# Autodesk Inventor assembly: 110033226_iam_12_船屋
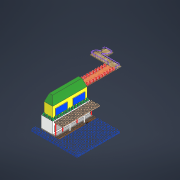
[picture p0: Inventor's stored thumbnail of the model, 180x180]
Saved by Autodesk Inventor 2022 (Build 260153000, 153)
## iProperties
Created: 2022-06-28
Part Number: 110033226_iam_12_船屋
Document SubType Name: Assembly
Designer: User
Author: User
## Documents named in this file (7)
- D:\D-disk\pomelo\大一\下學期\機械設計製圖\1100332260_LEGOproj_沒有公主城堡\110033226_iam_12_船屋.iam
- D:\D-disk\pomelo\大一\下學期\機械設計製圖\1100332260_LEGOproj_沒有公主城堡\110033226_ipt_47_船屋基地.ipt
- D:\D-disk\pomelo\大一\下學期\機械設計製圖\1100332260_LEGOproj_沒有公主城堡\110033226_ipt_48_船屋梁架.ipt
- D:\D-disk\pomelo\大一\下學期\機械設計製圖\1100332260_LEGOproj_沒有公主城堡\110033226_ipt_49_船屋主體.ipt
- D:\D-disk\pomelo\大一\下學期\機械設計製圖\1100332260_LEGOproj_沒有公主城堡\110033226_ipt_50_船屋圓柱.ipt
- D:\D-disk\pomelo\大一\下學期\機械設計製圖\1100332260_LEGOproj_沒有公主城堡\110033226_ipt_21_柵欄.ipt
- D:\D-disk\pomelo\大一\下學期\機械設計製圖\1100332260_LEGOproj_沒有公主城堡\110033226_ipt_04_小河.ipt
## Components (353 placed, 6 different names)
1. 110033226_ipt_48_船屋梁架:1 — 貼合:4, 貼合:5, 貼合:7
2. 110033226_ipt_49_船屋主體:1 — 貼合:6, 貼合:7, 貼合:11, 貼合:12, 貼合:13, 貼合:14, 貼合:15, 貼合:16, 貼合:17, 貼合:18, 貼合:19, 貼合:20, 貼合:21, 貼合:22, 貼合:23, 貼合:24, 貼合:25, 貼合:26, 貼合:27, 貼合:28, 貼合:29, 貼合:30, 貼合:31, 貼合:32, 貼合:33, 貼合:34
3. 110033226_ipt_21_柵欄:32 — 貼合:27, 貼合:28, 貼合:29, 角度:1
4. 110033226_ipt_47_船屋基地:1 — 貼合:1, 貼合:2, 貼合:3, 貼合:35, 貼合:36, 貼合:37, 貼合:38, 貼合:39, 貼合:40
5. 110033226_ipt_47_船屋基地:2 — 貼合:4, 貼合:5, 貼合:6, 貼合:8, 貼合:9, 貼合:10, 貼合:13, 貼合:14
6. 110033226_ipt_50_船屋圓柱:1 — 貼合:8, 貼合:9, 貼合:10
7. 110033226_ipt_50_船屋圓柱:2
8. 110033226_ipt_21_柵欄:1 — 貼合:11, 貼合:12
9. 110033226_ipt_21_柵欄:2
10. 110033226_ipt_21_柵欄:3
11. 110033226_ipt_21_柵欄:4
12. 110033226_ipt_21_柵欄:5
13. 110033226_ipt_21_柵欄:6
14. 110033226_ipt_21_柵欄:7
15. 110033226_ipt_21_柵欄:8
16. 110033226_ipt_21_柵欄:9
17. 110033226_ipt_21_柵欄:10
18. 110033226_ipt_21_柵欄:11
19. 110033226_ipt_21_柵欄:12
20. 110033226_ipt_21_柵欄:13
21. 110033226_ipt_21_柵欄:14 — 貼合:15, 貼合:16, 貼合:17
22. 110033226_ipt_21_柵欄:15
23. 110033226_ipt_21_柵欄:16
24. 110033226_ipt_21_柵欄:17
25. 110033226_ipt_21_柵欄:18
26. 110033226_ipt_21_柵欄:19
27. 110033226_ipt_21_柵欄:21 — 貼合:18, 貼合:19, 貼合:20
28. 110033226_ipt_21_柵欄:23
29. 110033226_ipt_21_柵欄:22 — 貼合:21, 貼合:22, 貼合:23
30. 110033226_ipt_21_柵欄:24
31. 110033226_ipt_21_柵欄:25
32. 110033226_ipt_21_柵欄:26
33. 110033226_ipt_21_柵欄:27
34. 110033226_ipt_21_柵欄:20 — 貼合:24, 貼合:25, 貼合:26
35. 110033226_ipt_21_柵欄:28
36. 110033226_ipt_21_柵欄:29
37. 110033226_ipt_21_柵欄:30
38. 110033226_ipt_21_柵欄:31 — 貼合:30, 貼合:31, 角度:1
39. 110033226_ipt_21_柵欄:33
40. 110033226_ipt_21_柵欄:34
41. 110033226_ipt_21_柵欄:35
42. 110033226_ipt_21_柵欄:36
43. 110033226_ipt_21_柵欄:37
44. 110033226_ipt_21_柵欄:38
45. 110033226_ipt_21_柵欄:39
46. 110033226_ipt_21_柵欄:40
47. 110033226_ipt_21_柵欄:41
48. 110033226_ipt_21_柵欄:42
49. 110033226_ipt_21_柵欄:43
50. 110033226_ipt_21_柵欄:44
51. 110033226_ipt_21_柵欄:45
52. 110033226_ipt_21_柵欄:46
53. 110033226_ipt_21_柵欄:47
54. 110033226_ipt_21_柵欄:48
55. 110033226_ipt_21_柵欄:49 — 貼合:32, 貼合:33, 貼合:34
56. 110033226_ipt_21_柵欄:50
57. 110033226_ipt_21_柵欄:51
58. 110033226_ipt_21_柵欄:52
59. 110033226_ipt_21_柵欄:53
60. 110033226_ipt_21_柵欄:54
61. 110033226_ipt_21_柵欄:55
62. 110033226_ipt_21_柵欄:56
63. 110033226_ipt_21_柵欄:57
64. 110033226_ipt_21_柵欄:58
65. 110033226_ipt_21_柵欄:59
66. 110033226_ipt_21_柵欄:60
67. 110033226_ipt_21_柵欄:61
68. 110033226_ipt_21_柵欄:62
69. 110033226_ipt_21_柵欄:63
70. 110033226_ipt_21_柵欄:64
71. 110033226_ipt_21_柵欄:65
72. 110033226_ipt_21_柵欄:66
73. 110033226_ipt_21_柵欄:67
74. 110033226_ipt_04_小河:2 — 貼合:36, 貼合:39, 貼合:40
75. 110033226_ipt_04_小河:29
76. 110033226_ipt_04_小河:30
77. 110033226_ipt_04_小河:31
78. 110033226_ipt_04_小河:32
79. 110033226_ipt_04_小河:33
80. 110033226_ipt_04_小河:34
81. 110033226_ipt_04_小河:35
82. 110033226_ipt_04_小河:36
83. 110033226_ipt_04_小河:37
84. 110033226_ipt_04_小河:38
85. 110033226_ipt_04_小河:39
86. 110033226_ipt_04_小河:40
87. 110033226_ipt_04_小河:41
88. 110033226_ipt_04_小河:42
89. 110033226_ipt_04_小河:43
90. 110033226_ipt_04_小河:44
91. 110033226_ipt_04_小河:45
92. 110033226_ipt_04_小河:46
93. 110033226_ipt_04_小河:47
94. 110033226_ipt_04_小河:48
95. 110033226_ipt_04_小河:49
96. 110033226_ipt_04_小河:50
97. 110033226_ipt_04_小河:51
98. 110033226_ipt_04_小河:52
99. 110033226_ipt_04_小河:53
100. 110033226_ipt_04_小河:54
101. 110033226_ipt_04_小河:55
102. 110033226_ipt_04_小河:56
103. 110033226_ipt_04_小河:57
104. 110033226_ipt_04_小河:58
105. 110033226_ipt_04_小河:59
106. 110033226_ipt_04_小河:60
107. 110033226_ipt_04_小河:61
108. 110033226_ipt_04_小河:62
109. 110033226_ipt_04_小河:63
110. 110033226_ipt_04_小河:64
111. 110033226_ipt_04_小河:65
112. 110033226_ipt_04_小河:66
113. 110033226_ipt_04_小河:67
114. 110033226_ipt_04_小河:68
115. 110033226_ipt_04_小河:69
116. 110033226_ipt_04_小河:70
117. 110033226_ipt_04_小河:71
118. 110033226_ipt_04_小河:72
119. 110033226_ipt_04_小河:73
120. 110033226_ipt_04_小河:74
121. 110033226_ipt_04_小河:75
122. 110033226_ipt_04_小河:76
123. 110033226_ipt_04_小河:77
124. 110033226_ipt_04_小河:78
125. 110033226_ipt_04_小河:79
126. 110033226_ipt_04_小河:80
127. 110033226_ipt_04_小河:81
128. 110033226_ipt_04_小河:82
129. 110033226_ipt_04_小河:83
130. 110033226_ipt_04_小河:84
131. 110033226_ipt_04_小河:85
132. 110033226_ipt_04_小河:86
133. 110033226_ipt_04_小河:87
134. 110033226_ipt_04_小河:88
135. 110033226_ipt_04_小河:89
136. 110033226_ipt_04_小河:90
137. 110033226_ipt_04_小河:91
138. 110033226_ipt_04_小河:1 — 貼合:35, 貼合:37, 貼合:38
139. 110033226_ipt_04_小河:3
140. 110033226_ipt_04_小河:4
141. 110033226_ipt_04_小河:5
142. 110033226_ipt_04_小河:6
143. 110033226_ipt_04_小河:7
144. 110033226_ipt_04_小河:8
145. 110033226_ipt_04_小河:9
146. 110033226_ipt_04_小河:10
147. 110033226_ipt_04_小河:11
148. 110033226_ipt_04_小河:12
149. 110033226_ipt_04_小河:13
150. 110033226_ipt_04_小河:14
151. 110033226_ipt_04_小河:15
152. 110033226_ipt_04_小河:16
153. 110033226_ipt_04_小河:17
154. 110033226_ipt_04_小河:18
155. 110033226_ipt_04_小河:19
156. 110033226_ipt_04_小河:20
157. 110033226_ipt_04_小河:21
158. 110033226_ipt_04_小河:22
159. 110033226_ipt_04_小河:23
160. 110033226_ipt_04_小河:24
161. 110033226_ipt_04_小河:25
162. 110033226_ipt_04_小河:26
163. 110033226_ipt_04_小河:27
164. 110033226_ipt_04_小河:28
165. 110033226_ipt_04_小河:92
166. 110033226_ipt_04_小河:93
167. 110033226_ipt_04_小河:94
168. 110033226_ipt_04_小河:95
169. 110033226_ipt_04_小河:96
170. 110033226_ipt_04_小河:97
171. 110033226_ipt_04_小河:98
172. 110033226_ipt_04_小河:99
173. 110033226_ipt_04_小河:100
174. 110033226_ipt_04_小河:101
175. 110033226_ipt_04_小河:102
176. 110033226_ipt_04_小河:103
177. 110033226_ipt_04_小河:104
178. 110033226_ipt_04_小河:105
179. 110033226_ipt_04_小河:106
180. 110033226_ipt_04_小河:107
181. 110033226_ipt_04_小河:108
182. 110033226_ipt_04_小河:109
183. 110033226_ipt_04_小河:110
184. 110033226_ipt_04_小河:111
185. 110033226_ipt_04_小河:112
186. 110033226_ipt_04_小河:113
187. 110033226_ipt_04_小河:114
188. 110033226_ipt_04_小河:115
189. 110033226_ipt_04_小河:116
190. 110033226_ipt_04_小河:117
191. 110033226_ipt_04_小河:118
192. 110033226_ipt_04_小河:119
193. 110033226_ipt_04_小河:120
194. 110033226_ipt_04_小河:121
195. 110033226_ipt_04_小河:122
196. 110033226_ipt_04_小河:123
197. 110033226_ipt_04_小河:124
198. 110033226_ipt_04_小河:125
199. 110033226_ipt_04_小河:126
200. 110033226_ipt_04_小河:127
201. 110033226_ipt_04_小河:128
202. 110033226_ipt_04_小河:129
203. 110033226_ipt_04_小河:130
204. 110033226_ipt_04_小河:131
205. 110033226_ipt_04_小河:132
206. 110033226_ipt_04_小河:133
207. 110033226_ipt_04_小河:134
208. 110033226_ipt_04_小河:135
209. 110033226_ipt_04_小河:136
210. 110033226_ipt_04_小河:137
211. 110033226_ipt_04_小河:138
212. 110033226_ipt_04_小河:139
213. 110033226_ipt_04_小河:140
214. 110033226_ipt_04_小河:141
215. 110033226_ipt_04_小河:142
216. 110033226_ipt_04_小河:143
217. 110033226_ipt_04_小河:144
218. 110033226_ipt_04_小河:145
219. 110033226_ipt_04_小河:146
220. 110033226_ipt_04_小河:147
221. 110033226_ipt_04_小河:148
222. 110033226_ipt_04_小河:149
223. 110033226_ipt_04_小河:150
224. 110033226_ipt_04_小河:151
225. 110033226_ipt_04_小河:152
226. 110033226_ipt_04_小河:153
227. 110033226_ipt_04_小河:154
228. 110033226_ipt_04_小河:155
229. 110033226_ipt_04_小河:156
230. 110033226_ipt_04_小河:157
231. 110033226_ipt_04_小河:158
232. 110033226_ipt_04_小河:159
233. 110033226_ipt_04_小河:160
234. 110033226_ipt_04_小河:161
235. 110033226_ipt_04_小河:162
236. 110033226_ipt_04_小河:163
237. 110033226_ipt_04_小河:164
238. 110033226_ipt_04_小河:165
239. 110033226_ipt_04_小河:166
240. 110033226_ipt_04_小河:167
241. 110033226_ipt_04_小河:168
242. 110033226_ipt_04_小河:169
243. 110033226_ipt_04_小河:170
244. 110033226_ipt_04_小河:171
245. 110033226_ipt_04_小河:172
246. 110033226_ipt_04_小河:173
247. 110033226_ipt_04_小河:174
248. 110033226_ipt_04_小河:175
249. 110033226_ipt_04_小河:176
250. 110033226_ipt_04_小河:177
251. 110033226_ipt_04_小河:178
252. 110033226_ipt_04_小河:179
253. 110033226_ipt_04_小河:180
254. 110033226_ipt_04_小河:181
255. 110033226_ipt_04_小河:182
256. 110033226_ipt_04_小河:183
257. 110033226_ipt_04_小河:184
258. 110033226_ipt_04_小河:185
259. 110033226_ipt_04_小河:186
260. 110033226_ipt_04_小河:187
261. 110033226_ipt_04_小河:188
262. 110033226_ipt_04_小河:189
263. 110033226_ipt_04_小河:190
264. 110033226_ipt_04_小河:191
265. 110033226_ipt_04_小河:192
266. 110033226_ipt_04_小河:193
267. 110033226_ipt_04_小河:194
268. 110033226_ipt_04_小河:195
269. 110033226_ipt_04_小河:196
270. 110033226_ipt_04_小河:197
271. 110033226_ipt_04_小河:198
272. 110033226_ipt_04_小河:199
273. 110033226_ipt_04_小河:200
274. 110033226_ipt_04_小河:201
275. 110033226_ipt_04_小河:202
276. 110033226_ipt_04_小河:203
277. 110033226_ipt_04_小河:204
278. 110033226_ipt_04_小河:205
279. 110033226_ipt_04_小河:206
280. 110033226_ipt_04_小河:207
281. 110033226_ipt_04_小河:208
282. 110033226_ipt_04_小河:209
283. 110033226_ipt_04_小河:210
284. 110033226_ipt_04_小河:211
285. 110033226_ipt_04_小河:212
286. 110033226_ipt_04_小河:213
287. 110033226_ipt_04_小河:214
288. 110033226_ipt_04_小河:215
289. 110033226_ipt_04_小河:216
290. 110033226_ipt_04_小河:217
291. 110033226_ipt_04_小河:218
292. 110033226_ipt_04_小河:219
293. 110033226_ipt_04_小河:220
294. 110033226_ipt_04_小河:221
295. 110033226_ipt_04_小河:222
296. 110033226_ipt_04_小河:223
297. 110033226_ipt_04_小河:224
298. 110033226_ipt_04_小河:225
299. 110033226_ipt_04_小河:226
300. 110033226_ipt_04_小河:227
301. 110033226_ipt_04_小河:228
302. 110033226_ipt_04_小河:229
303. 110033226_ipt_04_小河:230
304. 110033226_ipt_04_小河:231
305. 110033226_ipt_04_小河:232
306. 110033226_ipt_04_小河:233
307. 110033226_ipt_04_小河:234
308. 110033226_ipt_04_小河:235
309. 110033226_ipt_04_小河:236
310. 110033226_ipt_04_小河:237
311. 110033226_ipt_04_小河:238
312. 110033226_ipt_04_小河:239
313. 110033226_ipt_04_小河:240
314. 110033226_ipt_04_小河:241
315. 110033226_ipt_04_小河:242
316. 110033226_ipt_04_小河:243
317. 110033226_ipt_04_小河:244
318. 110033226_ipt_04_小河:245
319. 110033226_ipt_04_小河:246
320. 110033226_ipt_04_小河:247
321. 110033226_ipt_04_小河:248
322. 110033226_ipt_04_小河:249
323. 110033226_ipt_04_小河:250
324. 110033226_ipt_04_小河:251
325. 110033226_ipt_04_小河:252
326. 110033226_ipt_04_小河:253
327. 110033226_ipt_04_小河:254
328. 110033226_ipt_04_小河:255
329. 110033226_ipt_04_小河:256
330. 110033226_ipt_04_小河:257
331. 110033226_ipt_04_小河:258
332. 110033226_ipt_04_小河:259
333. 110033226_ipt_04_小河:260
334. 110033226_ipt_04_小河:261
335. 110033226_ipt_04_小河:262
336. 110033226_ipt_04_小河:263
337. 110033226_ipt_04_小河:264
338. 110033226_ipt_04_小河:265
339. 110033226_ipt_04_小河:266
340. 110033226_ipt_04_小河:267
341. 110033226_ipt_04_小河:268
342. 110033226_ipt_04_小河:269
343. 110033226_ipt_04_小河:270
344. 110033226_ipt_04_小河:271
345. 110033226_ipt_04_小河:272
346. 110033226_ipt_04_小河:273
347. 110033226_ipt_04_小河:274
348. 110033226_ipt_04_小河:275
349. 110033226_ipt_04_小河:276
350. 110033226_ipt_04_小河:277
351. 110033226_ipt_04_小河:278
352. 110033226_ipt_04_小河:279
353. 110033226_ipt_04_小河:280
## Component patterns: (2 elements, first: 110033226_ipt_47_船屋基地:1), (2 elements, first: 110033226_ipt_50_船屋圓柱:1), (13 elements, first: 110033226_ipt_21_柵欄:1), (6 elements, first: 110033226_ipt_21_柵欄:14), (2 elements, first: 110033226_ipt_21_柵欄:21), (5 elements, first: 110033226_ipt_21_柵欄:22), (4 elements, first: 110033226_ipt_21_柵欄:20), (17 elements, first: 110033226_ipt_21_柵欄:31), (19 elements, first: 110033226_ipt_21_柵欄:49), (2 elements), (8 elements), (32 elements, first: 110033226_ipt_04_小河:2), 元件陣列 11:2 (32 elements), (27 elements, first: 110033226_ipt_04_小河:1), 元件陣列 10:2 (27 elements), 元件陣列 10:3 (27 elements), 元件陣列 10:4 (27 elements), 元件陣列 10:5 (27 elements), 元件陣列 10:6 (27 elements), 元件陣列 10:7 (27 elements), 元件陣列 10:8 (27 elements)
## Relationships (41: Mate 40, Angle 1)
- 貼合:1 [Mate]: 110033226_ipt_47_船屋基地:1
- 貼合:2 [Mate]: 110033226_ipt_47_船屋基地:1
- 貼合:3 [Mate]: 110033226_ipt_47_船屋基地:1
- 貼合:4 [Mate]: 110033226_ipt_48_船屋梁架:1 ↔ 110033226_ipt_47_船屋基地:2
- 貼合:5 [Mate]: 110033226_ipt_48_船屋梁架:1 ↔ 110033226_ipt_47_船屋基地:2
- 貼合:6 [Mate]: 110033226_ipt_49_船屋主體:1 ↔ 110033226_ipt_47_船屋基地:2
- 貼合:7 [Mate]: 110033226_ipt_48_船屋梁架:1 ↔ 110033226_ipt_49_船屋主體:1
- 貼合:8 [Mate]: 110033226_ipt_47_船屋基地:2 ↔ 110033226_ipt_50_船屋圓柱:1
- 貼合:9 [Mate]: 110033226_ipt_47_船屋基地:2 ↔ 110033226_ipt_50_船屋圓柱:1
- 貼合:10 [Mate]: 110033226_ipt_47_船屋基地:2 ↔ 110033226_ipt_50_船屋圓柱:1
- 貼合:11 [Mate]: 110033226_ipt_49_船屋主體:1 ↔ 110033226_ipt_21_柵欄:1
- 貼合:12 [Mate]: 110033226_ipt_49_船屋主體:1 ↔ 110033226_ipt_21_柵欄:1
- 貼合:13 [Mate]: 110033226_ipt_49_船屋主體:1 ↔ 110033226_ipt_47_船屋基地:2
- 貼合:14 [Mate]: 110033226_ipt_49_船屋主體:1 ↔ 110033226_ipt_47_船屋基地:2
- 貼合:15 [Mate]: 110033226_ipt_49_船屋主體:1 ↔ 110033226_ipt_21_柵欄:14
- 貼合:16 [Mate]: 110033226_ipt_49_船屋主體:1 ↔ 110033226_ipt_21_柵欄:14
- 貼合:17 [Mate]: 110033226_ipt_49_船屋主體:1 ↔ 110033226_ipt_21_柵欄:14
- 貼合:18 [Mate]: 110033226_ipt_49_船屋主體:1 ↔ 110033226_ipt_21_柵欄:21
- 貼合:19 [Mate]: 110033226_ipt_49_船屋主體:1 ↔ 110033226_ipt_21_柵欄:21
- 貼合:20 [Mate]: 110033226_ipt_49_船屋主體:1 ↔ 110033226_ipt_21_柵欄:21
- 貼合:21 [Mate]: 110033226_ipt_49_船屋主體:1 ↔ 110033226_ipt_21_柵欄:22
- 貼合:22 [Mate]: 110033226_ipt_49_船屋主體:1 ↔ 110033226_ipt_21_柵欄:22
- 貼合:23 [Mate]: 110033226_ipt_49_船屋主體:1 ↔ 110033226_ipt_21_柵欄:22
- 貼合:24 [Mate]: 110033226_ipt_49_船屋主體:1 ↔ 110033226_ipt_21_柵欄:20
- 貼合:25 [Mate]: 110033226_ipt_49_船屋主體:1 ↔ 110033226_ipt_21_柵欄:20
- 貼合:26 [Mate]: 110033226_ipt_49_船屋主體:1 ↔ 110033226_ipt_21_柵欄:20
- 貼合:27 [Mate]: 110033226_ipt_49_船屋主體:1 ↔ 110033226_ipt_21_柵欄:32
- 貼合:28 [Mate]: 110033226_ipt_49_船屋主體:1 ↔ 110033226_ipt_21_柵欄:32
- 貼合:29 [Mate]: 110033226_ipt_49_船屋主體:1 ↔ 110033226_ipt_21_柵欄:32
- 貼合:30 [Mate]: 110033226_ipt_49_船屋主體:1 ↔ 110033226_ipt_21_柵欄:31
- 貼合:31 [Mate]: 110033226_ipt_49_船屋主體:1 ↔ 110033226_ipt_21_柵欄:31
- 角度:1 [Angle] (90 deg): 110033226_ipt_21_柵欄:32 ↔ 110033226_ipt_21_柵欄:31
- 貼合:32 [Mate]: 110033226_ipt_49_船屋主體:1 ↔ 110033226_ipt_21_柵欄:49
- 貼合:33 [Mate]: 110033226_ipt_49_船屋主體:1 ↔ 110033226_ipt_21_柵欄:49
- 貼合:34 [Mate]: 110033226_ipt_49_船屋主體:1 ↔ 110033226_ipt_21_柵欄:49
- 貼合:35 [Mate]: 110033226_ipt_47_船屋基地:1 ↔ 110033226_ipt_04_小河:1
- 貼合:36 [Mate]: 110033226_ipt_47_船屋基地:1 ↔ 110033226_ipt_04_小河:2
- 貼合:37 [Mate]: 110033226_ipt_47_船屋基地:1 ↔ 110033226_ipt_04_小河:1
- 貼合:38 [Mate]: 110033226_ipt_47_船屋基地:1 ↔ 110033226_ipt_04_小河:1
- 貼合:39 [Mate]: 110033226_ipt_47_船屋基地:1 ↔ 110033226_ipt_04_小河:2
- 貼合:40 [Mate]: 110033226_ipt_47_船屋基地:1 ↔ 110033226_ipt_04_小河:2
